# Autodesk Inventor assembly: Assembly2(gisdi)
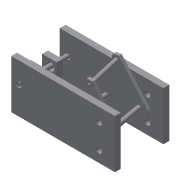
[picture p0: Inventor's stored thumbnail of the model, 180x180]
Saved by Autodesk Inventor 2019 (Build 230136000, 136)
## iProperties
Created: 2020-02-20
Part Number: Assembly2(gisdi)
Document SubType Name: Assembly
Designer: abhi bidari
Author: abhi bidari
## Documents named in this file (5)
- C:\Users\abhi bidari\Documents\Assembly2(gisdi).iam
- C:\Users\abhi bidari\Documents\abhi eng exp 3.ipt
- C:\Users\abhi bidari\Documents\abhi eng exp 2.ipt
- C:\Users\abhi bidari\Documents\assmebly 1(ahdfbvc).iam
- F:\autodesk diagrams\Abhi\exp 3.ipt
## Components (6 placed, 4 different names)
1. abhi eng exp 3:1 — Mate:1
2. abhi eng exp 3:2 — Rotational:1
3. abhi eng exp 2:1 — Rotational:1, Mate:1, Mate:4, Mate:5
4. assmebly 1(ahdfbvc):1 [sub-assembly]
5. exp 3:1 — Mate:5
6. exp 3:2 — Mate:4
## Relationships (4: Mate 3, RevoluteJoint 1)
- Rotational:1 [RevoluteJoint]: abhi eng exp 3:2 ↔ abhi eng exp 2:1
- Mate:1: abhi eng exp 3:1 ↔ abhi eng exp 2:1
- Mate:4: abhi eng exp 2:1 ↔ exp 3:2
- Mate:5: abhi eng exp 2:1 ↔ exp 3:1
